# Autodesk Inventor assembly: Elevator Motor Assembly_MIR1
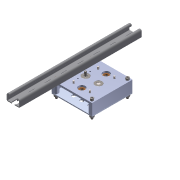
[picture p0: Inventor's stored thumbnail of the model, 180x180]
Saved by Autodesk Inventor 2015 (Build 190159000, 159)
## iProperties
Created: 2015-01-24
Part Number: Elevator Motor Assembly_MIR1
Document SubType Name: Assembly
Designer: Peter
Author: Peter
## Documents named in this file (3)
- C:\Users\Tanner\Documents\GitHub\FIRST-Team-1719-CAD-Team\2015 Robot CAD\Lifter Super Structure\Tower\Elevator Motor Assembly\Elevator Motor Assembly_MIR1.iam
- C:\Users\Tanner\Documents\GitHub\FIRST-Team-1719-CAD-Team\2015 Robot CAD\Lifter Super Structure\Tower\Elevator Motor Assembly\Andy Mark Tough Box_MIR1.iam
- C:\Users\Tanner\Documents\GitHub\FIRST-Team-1719-CAD-Team\2015 Robot CAD\Lifter Super Structure\Tower\H-Shaped-Assembly\Horizontal-Unistrut-Tower-Connector-15 w holes.ipt
## Components (2 placed, 2 different names)
1. Andy Mark Tough Box_MIR1:1 [sub-assembly] — Angle:1, Flush:1, Mate:1, Flush:2
2. Horizontal-Unistrut-Tower-Connector-15 w holes:1 — Angle:1, Flush:1, Mate:1, Flush:2
## Relationships (4: Flush 2, Angle 1, Mate 1)
- Angle:1 (0 deg): Andy Mark Tough Box_MIR1:1 ↔ Horizontal-Unistrut-Tower-Connector-15 w holes:1
- Flush:1 (127 mm): Andy Mark Tough Box_MIR1:1 ↔ Horizontal-Unistrut-Tower-Connector-15 w holes:1
- Mate:1: Andy Mark Tough Box_MIR1:1 ↔ Horizontal-Unistrut-Tower-Connector-15 w holes:1
- Flush:2 (12.7127 mm): Andy Mark Tough Box_MIR1:1 ↔ Horizontal-Unistrut-Tower-Connector-15 w holes:1
